# Autodesk Inventor assembly: Weldment
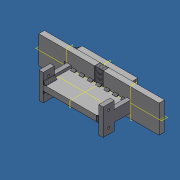
[picture p0: Inventor's stored thumbnail of the model, 180x180]
Saved by Autodesk Inventor 2022.4 (Build 264492010, 492A)
## iProperties
Created: 2006-01-12
Part Number: Weldment
Document SubType Name: Weldment
Designer: Administrator
Weld Material: Welded Steel Mild
Mass: 27441.4 g
Surface Area: 4421.87 cm^2
Volume: 3822.11 cm^3
Density: 7.17966 g/cm^3
CN_MASS: 27.44
Author: Administrator
## Documents named in this file (3)
- U:\Inventor 2022 Training\_Designer Training\Inventor 2022 - Advanced Assembly\Practice Files\Weldment.iam
- U:\Inventor 2022 Training\_Designer Training\Inventor 2022 - Advanced Assembly\Practice Files\Tbracket.ipt
- U:\Inventor 2022 Training\_Designer Training\Inventor 2022 - Advanced Assembly\Practice Files\base_support.ipt
## Components (6 placed, 2 different names)
1. base_support:1 — Mate:1, Flush:5, Flush:10, Mate:7
2. base_support:2 — Mate:1, Flush:5, Flush:10, Mate:2, Flush:3, Mate:6, Flush:11, Mate:8
3. base_support:3 — Mate:2, Flush:3, Mate:6
4. base_support:4 — Flush:11, Mate:7, Mate:8, Mate:9, Flush:12, Flush:13, Mate:10, Flush:14, Flush:15
5. Tbracket:1 — Mate:9, Flush:12, Flush:13
6. Tbracket:2 — Mate:10, Flush:14, Flush:15
## Relationships (15: Flush 8, Mate 7)
- Mate:1: base_support:1 ↔ base_support:2
- Flush:5: base_support:1 ↔ base_support:2
- Flush:10 (20 mm): base_support:1 ↔ base_support:2
- Mate:2: base_support:2 ↔ base_support:3
- Flush:3: base_support:2 ↔ base_support:3
- Flush:11: base_support:2 ↔ base_support:4
- Mate:6 (20 mm): base_support:2 ↔ base_support:3
- Mate:7: base_support:1 ↔ base_support:4
- Mate:8: base_support:2 ↔ base_support:4
- Mate:9: base_support:4 ↔ Tbracket:1
- Flush:12: base_support:4 ↔ Tbracket:1
- Flush:13: base_support:4 ↔ Tbracket:1
- Mate:10: base_support:4 ↔ Tbracket:2
- Flush:14: base_support:4 ↔ Tbracket:2
- Flush:15: base_support:4 ↔ Tbracket:2
